# Autodesk Inventor assembly: roboot
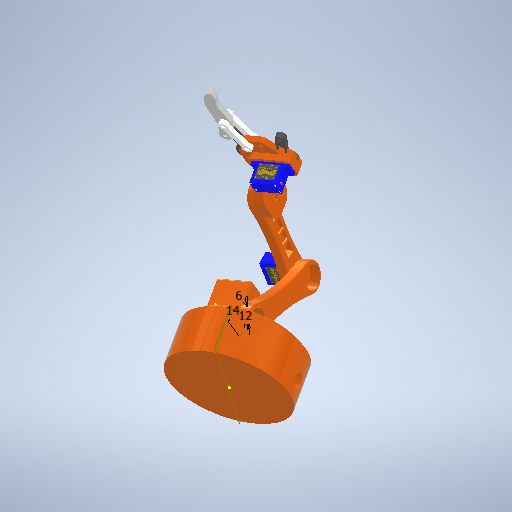
[picture p0: Inventor's stored thumbnail of the model, 512x512]
Saved by Autodesk Inventor 2025.2 (Build 292293000, 293)
## iProperties
Created: 2025-08-22
Part Number: roboot
Document SubType Name: Assembly
Designer: IGOR
Author: IGOR
## Documents named in this file (13)
- C:\Users\IGOR\OneDrive\Pulpit\chywtak 1\inventor\Nowy folder\roboot.iam
- C:\Users\IGOR\OneDrive\Pulpit\chywtak 1\inventor\Nowy folder\podstawa roobota.ipt
- C:\Users\IGOR\PycharmProjects\Downloads\Tower Pro MG90S Micro servo\Tower Pro MG90S Micro servo\Tower Pro MG90S Micro servo.ipt
- C:\Users\IGOR\PycharmProjects\Downloads\Four directed shoulder\Four directed shoulder\Four directed shoulder.ipt
- C:\Users\IGOR\OneDrive\Pulpit\chywtak 1\inventor\Nowy folder\baza.ipt
- C:\Users\IGOR\OneDrive\Pulpit\chywtak 1\inventor\Nowy folder\ramie dolne.ipt
- C:\Users\IGOR\PycharmProjects\Downloads\male_serwoo.iam
- C:\Users\IGOR\OneDrive\Pulpit\chywtak 1\inventor\Nowy folder\ramiegorav2.ipt
- C:\Users\IGOR\OneDrive\Pulpit\chywtak 1\inventor\Nowy folder\chwytka\Gripper base Ra\Gripper base Ra\Gripper base Ra.ipt
- C:\Users\IGOR\OneDrive\Pulpit\chywtak 1\inventor\Nowy folder\chwytka\Gear 1 Ra\Gear 1 Ra\Gear 1 Ra.ipt
- C:\Users\IGOR\OneDrive\Pulpit\chywtak 1\inventor\Nowy folder\chwytka\Gear 2 Ra\Gear 2 Ra\Gear 2 Ra.ipt
- C:\Users\IGOR\OneDrive\Pulpit\chywtak 1\inventor\Nowy folder\chwytka\Assembly Gripper Ra\Assembly Gripper Ra\Grip link 1 Ra.ipt
- C:\Users\IGOR\OneDrive\Pulpit\chywtak 1\inventor\Nowy folder\chwytka\grippeript.ipt
## Components (15 placed, 12 different names)
1. podstawa roobota:1 — Równoległe:1, Równoległe:2, Zestawiające:2, Zestawiające:3, Zestawiające:4
2. Tower Pro MG90S Micro servo:1 — Równoległe:1, Obrotowe:1, Równoległe:2, Zestawiające:2, Zestawiające:3, Zestawiające:4
3. Four directed shoulder:1 — Obrotowe:1, Sztywne:1
4. baza:1 — Sztywne:1, Równoległe:3, Zestawiające:5, Zestawiające:6
5. Tower Pro MG90S Micro servo:3 — Równoległe:3, Zestawiające:5, Zestawiające:6, Obrotowe:2
6. ramie dolne:1 — Obrotowe:2, Obrotowe:3
7. male_serwoo:1 [sub-assembly] — Obrotowe:3, Zestawiające:7, Zestawiające:8, Zestawiające:9
8. ramiegorav2:1 — Zestawiające:7, Zestawiające:8, Zestawiające:9, Zestawiające:10, Zestawiające:11, Obrotowe:4
9. Gripper base Ra:1 — Zestawiające:10, Zestawiające:11, Obrotowe:4, Zestawiające:12, Zestawiające:13, Zestawiające:14, Obrotowe:5, Obrotowe:7, Obrotowe:8
10. male_serwoo:3 [sub-assembly] — Zestawiające:12, Zestawiające:13, Zestawiające:14, Obrotowe:6
11. Gear 1 Ra:1 — Obrotowe:5, Obrotowe:11
12. Gear 2 Ra:1 — Obrotowe:6
13. Grip link 1 Ra:1 — Obrotowe:7, Zestawiające:15
14. Grip link 1 Ra:2 — Obrotowe:8, Zestawiające:16
15. grippeript:2 — Obrotowe:11, Zestawiające:15, Zestawiające:16
## Relationships (28: Mate 15, RevoluteJoint 9, Flush 3, WeldJoint 1)
- Równoległe:1 [Flush]: podstawa roobota:1 ↔ Tower Pro MG90S Micro servo:1
- Obrotowe:1 [RevoluteJoint] (1.5 mm): Tower Pro MG90S Micro servo:1 ↔ Four directed shoulder:1
- Równoległe:2 [Flush]: podstawa roobota:1 ↔ Tower Pro MG90S Micro servo:1
- Zestawiające:2 [Mate]: podstawa roobota:1 ↔ Tower Pro MG90S Micro servo:1
- Sztywne:1 [WeldJoint] (3 mm): Four directed shoulder:1 ↔ baza:1
- Zestawiające:3 [Mate]: podstawa roobota:1 ↔ Tower Pro MG90S Micro servo:1
- Zestawiające:4 [Mate]: podstawa roobota:1 ↔ Tower Pro MG90S Micro servo:1
- Równoległe:3 [Flush]: baza:1 ↔ Tower Pro MG90S Micro servo:3
- Zestawiające:5 [Mate] (1 mm): baza:1 ↔ Tower Pro MG90S Micro servo:3
- Zestawiające:6 [Mate] (7 mm): baza:1 ↔ Tower Pro MG90S Micro servo:3
- Obrotowe:2 [RevoluteJoint] (1 mm): Tower Pro MG90S Micro servo:3 ↔ ramie dolne:1
- Obrotowe:3 [RevoluteJoint]: ramie dolne:1 ↔ male_serwoo:1
- Zestawiające:7 [Mate]: male_serwoo:1 ↔ ramiegorav2:1
- Zestawiające:8 [Mate]: male_serwoo:1 ↔ ramiegorav2:1
- Zestawiające:9 [Mate]: male_serwoo:1 ↔ ramiegorav2:1
- Zestawiające:10 [Mate]: ramiegorav2:1 ↔ Gripper base Ra:1
- Zestawiające:11 [Mate]: ramiegorav2:1 ↔ Gripper base Ra:1
- Obrotowe:4 [RevoluteJoint]: ramiegorav2:1 ↔ Gripper base Ra:1
- Zestawiające:12 [Mate]: Gripper base Ra:1 ↔ male_serwoo:3
- Zestawiające:13 [Mate]: Gripper base Ra:1 ↔ male_serwoo:3
- Zestawiające:14 [Mate]: Gripper base Ra:1 ↔ male_serwoo:3
- Obrotowe:5 [RevoluteJoint]: Gripper base Ra:1 ↔ Gear 1 Ra:1
- Obrotowe:6 [RevoluteJoint] (-1 mm): male_serwoo:3 ↔ Gear 2 Ra:1
- Obrotowe:7 [RevoluteJoint]: Gripper base Ra:1 ↔ Grip link 1 Ra:1
- Obrotowe:8 [RevoluteJoint]: Gripper base Ra:1 ↔ Grip link 1 Ra:2
- Obrotowe:11 [RevoluteJoint]: Gear 1 Ra:1 ↔ grippeript:2
- Zestawiające:15 [Mate]: Grip link 1 Ra:1 ↔ grippeript:2
- Zestawiające:16 [Mate]: Grip link 1 Ra:2 ↔ grippeript:2
